# Autodesk Inventor assembly: front shell
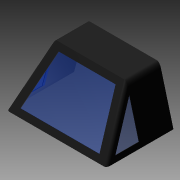
[picture p0: Inventor's stored thumbnail of the model, 180x180]
Saved by Autodesk Inventor 2012 (Build 160160000, 160)
## iProperties
Created: 2011-12-02
Part Number: front shell
Document SubType Name: Assembly
Designer: Antonella
Author: Antonella
## Documents named in this file (4)
- C:\Users\Antonella\Documents\GCC Robotics 2012 - Mechanical\Robot 2.0\Weatherproofing Shell\front shell.iam
- C:\Users\Antonella\Documents\GCC Robotics 2012 - Mechanical\Robot 2.0\Weatherproofing Shell\front shell.ipt
- C:\Users\Antonella\Documents\GCC Robotics 2012 - Mechanical\Robot 2.0\Weatherproofing Shell\front window.ipt
- C:\Users\Antonella\Documents\GCC Robotics 2012 - Mechanical\Robot 2.0\Weatherproofing Shell\side window.ipt
## Components (4 placed, 3 different names)
1. front shell:1 — Mate:1, Flush:1, Mate:2, Mate:3, Mate:4, Mate:5, Mate:6, Mate:7, Mate:8
2. front window:1 — Mate:1, Flush:1, Mate:2
3. side window:1 — Mate:6, Mate:7, Mate:8
4. side window:2 — Mate:3, Mate:4, Mate:5
## Relationships (9: Mate 8, Flush 1)
- Mate:1: front shell:1 ↔ front window:1
- Flush:1: front shell:1 ↔ front window:1
- Mate:2 (-1.5875 mm): front shell:1 ↔ front window:1
- Mate:3: front shell:1 ↔ side window:2
- Mate:4 (-12.7 mm): front shell:1 ↔ side window:2
- Mate:5: front shell:1 ↔ side window:2
- Mate:6: front shell:1 ↔ side window:1
- Mate:7 (12.7 mm): front shell:1 ↔ side window:1
- Mate:8: front shell:1 ↔ side window:1
